# Autodesk Inventor assembly: v1
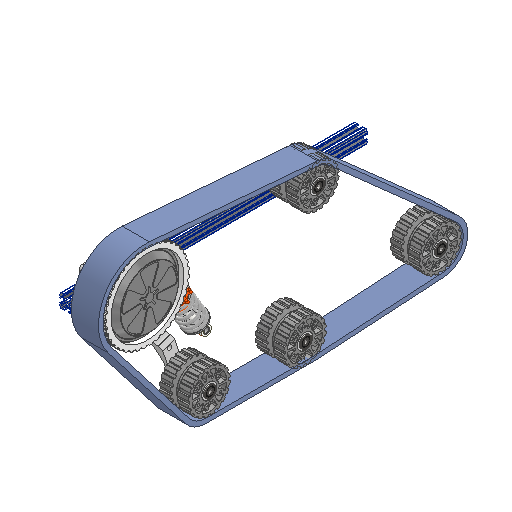
[picture p0: Inventor's stored thumbnail of the model, 512x512]
Saved by Autodesk Inventor 2025 (Build 290162000, 162)
## iProperties
Created: 2024-06-21
Part Number: v1
Document SubType Name: Assembly
Designer: derm
Mass: 3679.05 g
Surface Area: 9631.1 cm^2
Volume: 3232.7 cm^3
Density: 1.13807 g/cm^3
Author: derm
## Documents named in this file (16)
- C:\Users\derm\Desktop\puppycat\v1.iam
- C:\Users\derm\Desktop\puppycat\moteur hoverboard\hoverboard_motor_assembly\hoverboard_motor_assembly.ipt
- C:\Users\derm\Desktop\puppycat\am-3298a 20 tooth Molded Tank Pulley Half Rev4\am-3298a 20 tooth Molded Tank Pulley Half Rev4.ipt
- C:\Users\derm\Desktop\puppycat\6495K814_Timing Belt Pulley\6495K814_Timing Belt Pulley.ipt
- C:\Users\derm\Desktop\puppycat\6495K821_Timing Belt Pulley\6495K821_Timing Belt Pulley.ipt
- C:\Users\derm\Desktop\puppycat\hoverboardPulleyAdapter.ipt
- C:\Users\derm\Desktop\puppycat\6495K822_Timing Belt Pulley\6495K822_Timing Belt Pulley.ipt
- C:\Users\derm\Desktop\puppycat\6082rsBearing.ipt
- C:\Users\derm\Desktop\puppycat\am3298_bearing_adapter.ipt
- C:\Users\derm\Desktop\puppycat\beltConifgV1.ipt
- C:\Users\derm\Desktop\puppycat\stairs\stairs.ipt
- C:\Users\derm\Desktop\puppycat\trackBase.ipt
- C:\Users\derm\Desktop\puppycat\125 mm Bike Rear Shock Absorber\125 mm Bike Rear Shock Absorber.ipt
- C:\Users\derm\Desktop\puppycat\swingarmBase.ipt
- C:\Users\derm\Desktop\puppycat\swingarmV1.ipt
- C:\Users\derm\Desktop\puppycat\hoverboardMotorMount.ipt
## Components (38 placed, 15 different names)
1. hoverboard_motor_assembly:1 — Mate:6, Mate:8, Mate:52, Flush:4, Mate:67
2. am-3298a 20 tooth Molded Tank Pulley Half Rev4:1 — Mate:1, Mate:2, Mate:3, Mate:13, Mate:14
3. am-3298a 20 tooth Molded Tank Pulley Half Rev4:2 — Mate:1, Mate:2, Mate:3, Mate:10, Mate:11, Mate:28
4. 6495K814_Timing Belt Pulley:1
5. 6495K821_Timing Belt Pulley:1 — Mate:5, Flush:1
6. hoverboardPulleyAdapter:1 — Mate:5, Flush:1, Mate:6, Mate:7, Mate:8, Mate:28, Mate:29
7. 6495K822_Timing Belt Pulley:1 — Mate:7
8. 6082rsBearing:1 — Mate:15, Mate:16, Mate:58, Mate:64
9. 6082rsBearing:2 — Mate:9, Mate:11, Mate:12
10. am3298_bearing_adapter:1 — Mate:9, Mate:10, Mate:12
11. am3298_bearing_adapter:2 — Mate:13, Mate:14, Mate:15, Mate:16
12. am-3298a 20 tooth Molded Tank Pulley Half Rev4:3
13. am-3298a 20 tooth Molded Tank Pulley Half Rev4:4 — Mate:29, Flush:2
14. 6082rsBearing:3
15. 6082rsBearing:4
16. am3298_bearing_adapter:3
17. am3298_bearing_adapter:4
18. am-3298a 20 tooth Molded Tank Pulley Half Rev4:5
19. am-3298a 20 tooth Molded Tank Pulley Half Rev4:6 — Flush:2, Flush:3
20. 6082rsBearing:5
21. 6082rsBearing:6
22. am3298_bearing_adapter:5
23. am3298_bearing_adapter:6
24. am-3298a 20 tooth Molded Tank Pulley Half Rev4:7
25. am-3298a 20 tooth Molded Tank Pulley Half Rev4:8 — Flush:3
26. 6082rsBearing:7
27. 6082rsBearing:8
28. am3298_bearing_adapter:7
29. am3298_bearing_adapter:8
30. beltConifgV1:1
31. stairs:1
32. trackBase:1 — Mate:52, Flush:4, Mate:53, Mate:57, Angle:1
33. 125 mm Bike Rear Shock Absorber:1 — Mate:63, Mate:65, Mate:66
34. swingarmBase:1 — Mate:53, Mate:55, Mate:56, Mate:57, Mate:60, Mate:61, Mate:63, Mate:65, Mate:66
35. 6082rsBearing:9 — Mate:55, Mate:56, Mate:59
36. swingarmV1:1 — Mate:58, Mate:59, Mate:62, Mate:64
37. 6082rsBearing:10 — Mate:60, Mate:61, Mate:62
38. hoverboardMotorMount:1 — Mate:67, Angle:1
## Relationships (70: Mate 65, Flush 4, Angle 1)
- Mate:1: am-3298a 20 tooth Molded Tank Pulley Half Rev4:1 ↔ am-3298a 20 tooth Molded Tank Pulley Half Rev4:2
- Mate:2: am-3298a 20 tooth Molded Tank Pulley Half Rev4:1 ↔ am-3298a 20 tooth Molded Tank Pulley Half Rev4:2
- Mate:3: am-3298a 20 tooth Molded Tank Pulley Half Rev4:1 ↔ am-3298a 20 tooth Molded Tank Pulley Half Rev4:2
- Mate:5: 6495K821_Timing Belt Pulley:1 ↔ hoverboardPulleyAdapter:1
- Flush:1: 6495K821_Timing Belt Pulley:1 ↔ hoverboardPulleyAdapter:1
- Mate:6: hoverboard_motor_assembly:1 ↔ hoverboardPulleyAdapter:1
- Mate:7: hoverboardPulleyAdapter:1 ↔ 6495K822_Timing Belt Pulley:1
- Mate:8: hoverboard_motor_assembly:1 ↔ hoverboardPulleyAdapter:1
- Mate:9: 6082rsBearing:2 ↔ am3298_bearing_adapter:1
- Mate:10: am-3298a 20 tooth Molded Tank Pulley Half Rev4:2 ↔ am3298_bearing_adapter:1
- Mate:11: am-3298a 20 tooth Molded Tank Pulley Half Rev4:2 ↔ 6082rsBearing:2
- Mate:12: 6082rsBearing:2 ↔ am3298_bearing_adapter:1
- Mate:13: am-3298a 20 tooth Molded Tank Pulley Half Rev4:1 ↔ am3298_bearing_adapter:2
- Mate:14: am-3298a 20 tooth Molded Tank Pulley Half Rev4:1 ↔ am3298_bearing_adapter:2
- Mate:15: 6082rsBearing:1 ↔ am3298_bearing_adapter:2
- Mate:16: 6082rsBearing:1 ↔ am3298_bearing_adapter:2
- [Mate]: am-3298a 20 tooth Molded Tank Pulley Half Rev4:3 ↔ am-3298a 20 tooth Molded Tank Pulley Half Rev4:4
- [Mate]: am-3298a 20 tooth Molded Tank Pulley Half Rev4:3 ↔ am-3298a 20 tooth Molded Tank Pulley Half Rev4:4
- [Mate]: am-3298a 20 tooth Molded Tank Pulley Half Rev4:3 ↔ am-3298a 20 tooth Molded Tank Pulley Half Rev4:4
- [Mate]: 6082rsBearing:4 ↔ am3298_bearing_adapter:3
- [Mate]: am-3298a 20 tooth Molded Tank Pulley Half Rev4:4 ↔ am3298_bearing_adapter:3
- [Mate]: am-3298a 20 tooth Molded Tank Pulley Half Rev4:4 ↔ 6082rsBearing:4
- [Mate]: 6082rsBearing:4 ↔ am3298_bearing_adapter:3
- [Mate]: am-3298a 20 tooth Molded Tank Pulley Half Rev4:3 ↔ am3298_bearing_adapter:4
- [Mate]: am-3298a 20 tooth Molded Tank Pulley Half Rev4:3 ↔ am3298_bearing_adapter:4
- [Mate]: 6082rsBearing:3 ↔ am3298_bearing_adapter:4
- [Mate]: 6082rsBearing:3 ↔ am3298_bearing_adapter:4
- Mate:28: am-3298a 20 tooth Molded Tank Pulley Half Rev4:2 ↔ hoverboardPulleyAdapter:1
- Mate:29: hoverboardPulleyAdapter:1 ↔ am-3298a 20 tooth Molded Tank Pulley Half Rev4:4
- [Mate]: am-3298a 20 tooth Molded Tank Pulley Half Rev4:5 ↔ am-3298a 20 tooth Molded Tank Pulley Half Rev4:6
- [Mate]: am-3298a 20 tooth Molded Tank Pulley Half Rev4:5 ↔ am-3298a 20 tooth Molded Tank Pulley Half Rev4:6
- [Mate]: am-3298a 20 tooth Molded Tank Pulley Half Rev4:5 ↔ am-3298a 20 tooth Molded Tank Pulley Half Rev4:6
- [Mate]: 6082rsBearing:6 ↔ am3298_bearing_adapter:5
- [Mate]: am-3298a 20 tooth Molded Tank Pulley Half Rev4:6 ↔ am3298_bearing_adapter:5
- [Mate]: am-3298a 20 tooth Molded Tank Pulley Half Rev4:6 ↔ 6082rsBearing:6
- [Mate]: 6082rsBearing:6 ↔ am3298_bearing_adapter:5
- [Mate]: am-3298a 20 tooth Molded Tank Pulley Half Rev4:5 ↔ am3298_bearing_adapter:6
- [Mate]: am-3298a 20 tooth Molded Tank Pulley Half Rev4:5 ↔ am3298_bearing_adapter:6
- [Mate]: 6082rsBearing:5 ↔ am3298_bearing_adapter:6
- [Mate]: 6082rsBearing:5 ↔ am3298_bearing_adapter:6
- Flush:2: am-3298a 20 tooth Molded Tank Pulley Half Rev4:4 ↔ am-3298a 20 tooth Molded Tank Pulley Half Rev4:6
- [Mate]: am-3298a 20 tooth Molded Tank Pulley Half Rev4:7 ↔ am-3298a 20 tooth Molded Tank Pulley Half Rev4:8
- [Mate]: am-3298a 20 tooth Molded Tank Pulley Half Rev4:7 ↔ am-3298a 20 tooth Molded Tank Pulley Half Rev4:8
- [Mate]: am-3298a 20 tooth Molded Tank Pulley Half Rev4:7 ↔ am-3298a 20 tooth Molded Tank Pulley Half Rev4:8
- [Mate]: 6082rsBearing:8 ↔ am3298_bearing_adapter:7
- [Mate]: am-3298a 20 tooth Molded Tank Pulley Half Rev4:8 ↔ am3298_bearing_adapter:7
- [Mate]: am-3298a 20 tooth Molded Tank Pulley Half Rev4:8 ↔ 6082rsBearing:8
- [Mate]: 6082rsBearing:8 ↔ am3298_bearing_adapter:7
- [Mate]: am-3298a 20 tooth Molded Tank Pulley Half Rev4:7 ↔ am3298_bearing_adapter:8
- [Mate]: am-3298a 20 tooth Molded Tank Pulley Half Rev4:7 ↔ am3298_bearing_adapter:8
- [Mate]: 6082rsBearing:7 ↔ am3298_bearing_adapter:8
- [Mate]: 6082rsBearing:7 ↔ am3298_bearing_adapter:8
- Flush:3: am-3298a 20 tooth Molded Tank Pulley Half Rev4:6 ↔ am-3298a 20 tooth Molded Tank Pulley Half Rev4:8
- Mate:52: hoverboard_motor_assembly:1 ↔ trackBase:1
- Flush:4 (-12.7 mm): hoverboard_motor_assembly:1 ↔ trackBase:1
- Mate:53: trackBase:1 ↔ swingarmBase:1
- Mate:55: swingarmBase:1 ↔ 6082rsBearing:9
- Mate:56: swingarmBase:1 ↔ 6082rsBearing:9
- Mate:57: trackBase:1 ↔ swingarmBase:1
- Mate:58: 6082rsBearing:1 ↔ swingarmV1:1
- Mate:59: 6082rsBearing:9 ↔ swingarmV1:1
- Mate:60: swingarmBase:1 ↔ 6082rsBearing:10
- Mate:61: swingarmBase:1 ↔ 6082rsBearing:10
- Mate:62: swingarmV1:1 ↔ 6082rsBearing:10
- Mate:63: 125 mm Bike Rear Shock Absorber:1 ↔ swingarmBase:1
- Mate:64: 6082rsBearing:1 ↔ swingarmV1:1
- Mate:65: 125 mm Bike Rear Shock Absorber:1 ↔ swingarmBase:1
- Mate:66: 125 mm Bike Rear Shock Absorber:1 ↔ swingarmBase:1
- Mate:67: hoverboard_motor_assembly:1 ↔ hoverboardMotorMount:1
- Angle:1 (0 deg): trackBase:1 ↔ hoverboardMotorMount:1
## Named parameters: d17_d10 = 0 mm, d18_d11 = 0 mm, d19_d12 = 0 mm, d20_d13 = 0 mm, d21_d14 = 0 mm, d22_d15 = 0 mm, d23_d16 = 0 mm, d24_d0 = 0 mm, d25_d1 = 0 mm, d26_d2 = 0 mm, d27_d9 = 0 mm, d30_d17_d10 = 0 mm, d31_d18_d11 = 0 mm, d32_d19_d12 = 0 mm, d33_d20_d13 = 0 mm, d34_d21_d14 = 0 mm, d35_d22_d15 = 0 mm, d36_d23_d16 = 0 mm, d37_d24_d0 = 0 mm, d38_d25_d1 = 0 mm, d39_d26_d2 = 0 mm, d40_d27_d9 = 0 mm, d42_d30_d17_d10 = 0 mm, d43_d31_d18_d11 = 0 mm, d44_d32_d19_d12 = 0 mm, d45_d33_d20_d13 = 0 mm, d46_d34_d21_d14 = 0 mm, d47_d35_d22_d15 = 0 mm, d48_d36_d23_d16 = 0 mm, d49_d37_d24_d0 = 0 mm, d50_d38_d25_d1 = 0 mm, d51_d39_d26_d2 = 0 mm, d52_d40_d27_d9 = 0 mm
